# Autodesk Inventor assembly: TruckBaseplate
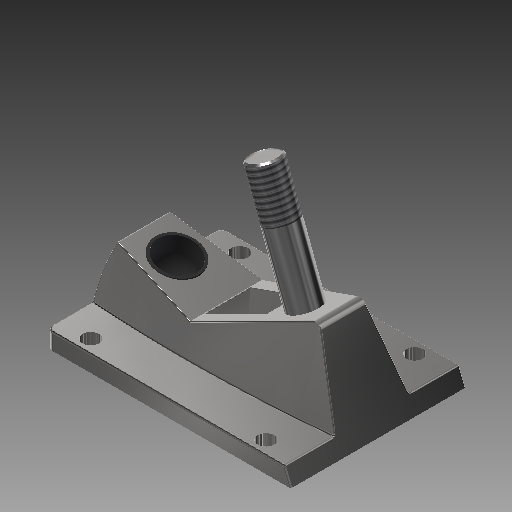
[picture p0: Inventor's stored thumbnail of the model, 512x512]
Saved by Autodesk Inventor 2019 (Build 230136000, 136)
## iProperties
Created: 2020-12-10
Part Number: TruckBaseplate
Document SubType Name: Assembly
Designer: Anass Hamdi
Author: Anass Hamdi
## Documents named in this file (4)
- C:\Users\Anass Hamdi\OneDrive - Vrije Universiteit Brussel\Documenten\Inventor\Anass Hamdi Project\TruckBaseplate.iam
- C:\Users\Anass Hamdi\OneDrive - Vrije Universiteit Brussel\Documenten\Inventor\Anass Hamdi Project\Kingpin_Bolt.ipt
- C:\Users\Anass Hamdi\OneDrive - Vrije Universiteit Brussel\Documenten\Inventor\Anass Hamdi Project\PivotCup.ipt
- C:\Users\Anass Hamdi\OneDrive - Vrije Universiteit Brussel\Documenten\Inventor\Anass Hamdi Project\Truck_Baseplate.ipt
## Components (3 placed, 3 different names)
1. Kingpin_Bolt:1 — Rigid:2
2. PivotCup:1 — Rigid:1
3. Truck_Baseplate:1 — Rigid:1, Rigid:2
## Relationships (2: WeldJoint 2)
- Rigid:1 [WeldJoint]: PivotCup:1 ↔ Truck_Baseplate:1
- Rigid:2 [WeldJoint]: Kingpin_Bolt:1 ↔ Truck_Baseplate:1
